# Autodesk Inventor assembly: assembly
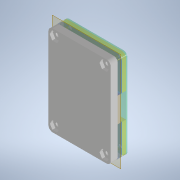
[picture p0: Inventor's stored thumbnail of the model, 180x180]
Saved by Autodesk Inventor 2021.2 (Build 252289000, 289)
## iProperties
Created: 2021-11-19
Part Number: assembly
Document SubType Name: Assembly
Designer: kanad
Author: kanad
## Documents named in this file (6)
- D:\Projects\IT\ok_pad\assembly.iam
- D:\Projects\IT\ok_pad\3dmodels\plate.ipt
- D:\Projects\IT\ok_pad\3dmodels\level1_up.ipt
- D:\Projects\IT\ok_pad\3dmodels\level2_up.ipt
- D:\Projects\IT\ok_pad\3dmodels\level3_up.ipt
- D:\Projects\IT\ok_pad\3dmodels\bottom.ipt
## Components (5 placed, 5 different names)
1. plate:1 — Заподлицо:1
2. level1_up:1 — Заподлицо:1, Заподлицо:2, Заподлицо:4, Заподлицо:5
3. level2_up:1 — Заподлицо:2, Заподлицо:3
4. level3_up:1 — Заподлицо:3
5. bottom:1 — Заподлицо:4, Заподлицо:5
## Relationships (5: Flush 5)
- Заподлицо:1 [Flush]: plate:1 ↔ level1_up:1
- Заподлицо:2 [Flush]: level1_up:1 ↔ level2_up:1
- Заподлицо:3 [Flush]: level2_up:1 ↔ level3_up:1
- Заподлицо:4 [Flush]: level1_up:1 ↔ bottom:1
- Заподлицо:5 [Flush]: level1_up:1 ↔ bottom:1
